# Autodesk Inventor assembly: stand2
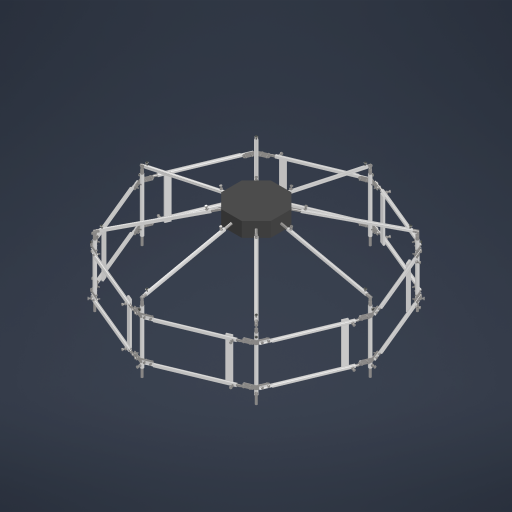
[picture p0: Inventor's stored thumbnail of the model, 512x512]
Saved by Autodesk Inventor 2023 (Build 270158000, 158)
## iProperties
Created: 2022-05-01
Part Number: stand2
Document SubType Name: Assembly
Designer: Norbert Ligas
stand_diameter: 400,000 mm
Author: Norbert Ligas
## Documents named in this file (3)
- C:\Users\norbe\Repozytoria\NormalMapScanner\stand_construction\stand.iam
- C:\Users\norbe\Repozytoria\NormalMapScanner\stand_construction\parts\leg_connector_arm.iam
- C:\Users\norbe\Repozytoria\NormalMapScanner\stand_construction\parts\board_case.ipt
## Components (9 placed, 2 different names)
1. board_case:1 — Angle:4, Mate:8, Mate:9, Mate:13, Mate:17, Mate:21, Mate:25, Mate:31, Mate:36, Mate:41
2. leg_connector_arm:1 [sub-assembly] — Flush:1, Flush:2, Mate:9, Mate:10, Mate:11, Mate:12, Tangent:1, Tangent:8, Mate:42, Mate:43
3. leg_connector_arm:2 [sub-assembly] — Mate:10, Mate:11, Mate:12, Tangent:1, Mate:13, Flush:3, Flush:4, Mate:14, Mate:15, Mate:16, Tangent:2
4. leg_connector_arm:3 [sub-assembly] — Mate:14, Mate:15, Mate:16, Tangent:2, Flush:5, Flush:6, Mate:17, Mate:18, Mate:19, Mate:20, Tangent:3
5. leg_connector_arm:4 [sub-assembly] — Mate:18, Mate:19, Mate:20, Tangent:3, Mate:21, Flush:7, Flush:8, Tangent:4, Mate:22, Mate:23, Mate:24
6. leg_connector_arm:5 [sub-assembly] — Tangent:4, Mate:22, Mate:23, Mate:24, Mate:25, Flush:9, Mate:26, Tangent:5, Mate:28, Mate:29, Mate:30
7. leg_connector_arm:6 [sub-assembly] — Tangent:5, Mate:27, Flush:10, Mate:28, Mate:29, Mate:30, Mate:31, Tangent:6, Mate:33, Mate:34, Mate:35
8. leg_connector_arm:7 [sub-assembly] — Mate:32, Flush:11, Tangent:6, Mate:33, Mate:34, Mate:35, Mate:36, Mate:38, Mate:39, Mate:40
9. leg_connector_arm:8 [sub-assembly] — Flush:12, Mate:37, Mate:38, Mate:39, Mate:40, Mate:41, Tangent:8, Mate:42, Mate:43
## Relationships (60: Mate 38, Flush 12, Tangent 7, Angle 3)
- Mate:3
- Angle:1 (45 deg)
- Mate:5
- Angle:3 (135 deg)
- Angle:4 (0 deg): board_case:1
- Mate:8: board_case:1
- Flush:1: leg_connector_arm:1
- Flush:2: leg_connector_arm:1
- Mate:9: board_case:1 ↔ leg_connector_arm:1
- Mate:10: leg_connector_arm:1 ↔ leg_connector_arm:2
- Mate:11: leg_connector_arm:1 ↔ leg_connector_arm:2
- Mate:12: leg_connector_arm:1 ↔ leg_connector_arm:2
- Tangent:1: leg_connector_arm:1 ↔ leg_connector_arm:2
- Mate:13: board_case:1 ↔ leg_connector_arm:2
- Flush:3: leg_connector_arm:2
- Flush:4: leg_connector_arm:2
- Mate:14: leg_connector_arm:2 ↔ leg_connector_arm:3
- Mate:15: leg_connector_arm:2 ↔ leg_connector_arm:3
- Mate:16: leg_connector_arm:2 ↔ leg_connector_arm:3
- Tangent:2: leg_connector_arm:2 ↔ leg_connector_arm:3
- Flush:5: leg_connector_arm:3
- Flush:6: leg_connector_arm:3
- Mate:17: board_case:1 ↔ leg_connector_arm:3
- Mate:18: leg_connector_arm:3 ↔ leg_connector_arm:4
- Mate:19: leg_connector_arm:3 ↔ leg_connector_arm:4
- Mate:20: leg_connector_arm:3 ↔ leg_connector_arm:4
- Tangent:3: leg_connector_arm:3 ↔ leg_connector_arm:4
- Mate:21: board_case:1 ↔ leg_connector_arm:4
- Flush:7: leg_connector_arm:4
- Flush:8: leg_connector_arm:4
- Tangent:4: leg_connector_arm:4 ↔ leg_connector_arm:5
- Mate:22: leg_connector_arm:4 ↔ leg_connector_arm:5
- Mate:23: leg_connector_arm:4 ↔ leg_connector_arm:5
- Mate:24: leg_connector_arm:4 ↔ leg_connector_arm:5
- Mate:25: board_case:1 ↔ leg_connector_arm:5
- Flush:9: leg_connector_arm:5
- Mate:26: leg_connector_arm:5
- Tangent:5: leg_connector_arm:5 ↔ leg_connector_arm:6
- Mate:27: leg_connector_arm:6
- Flush:10: leg_connector_arm:6
- Mate:28: leg_connector_arm:5 ↔ leg_connector_arm:6
- Mate:29: leg_connector_arm:5 ↔ leg_connector_arm:6
- Mate:30: leg_connector_arm:5 ↔ leg_connector_arm:6
- Mate:31: board_case:1 ↔ leg_connector_arm:6
- Mate:32: leg_connector_arm:7
- Flush:11: leg_connector_arm:7
- Tangent:6: leg_connector_arm:6 ↔ leg_connector_arm:7
- Mate:33: leg_connector_arm:6 ↔ leg_connector_arm:7
- Mate:34: leg_connector_arm:6 ↔ leg_connector_arm:7
- Mate:35: leg_connector_arm:6 ↔ leg_connector_arm:7
- Mate:36: board_case:1 ↔ leg_connector_arm:7
- Flush:12: leg_connector_arm:8
- Mate:37: leg_connector_arm:8
- Mate:38: leg_connector_arm:7 ↔ leg_connector_arm:8
- Mate:39: leg_connector_arm:7 ↔ leg_connector_arm:8
- Mate:40: leg_connector_arm:7 ↔ leg_connector_arm:8
- Mate:41: board_case:1 ↔ leg_connector_arm:8
- Tangent:8: leg_connector_arm:1 ↔ leg_connector_arm:8
- Mate:42: leg_connector_arm:1 ↔ leg_connector_arm:8
- Mate:43: leg_connector_arm:1 ↔ leg_connector_arm:8
